# Autodesk Inventor assembly: robot
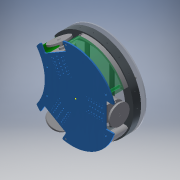
[picture p0: Inventor's stored thumbnail of the model, 180x180]
Saved by Autodesk Inventor 2016 (Build 200138000, 138)
## iProperties
Created: 2015-08-21
Part Number: robot
Document SubType Name: Assembly
Designer: TFHulbert
Author: TFHulbert
## Documents named in this file (11)
- C:\Users\Hulbert Office\Dropbox\SHF Robotics\robot.iam
- C:\Users\Hulbert Office\Dropbox\SHF Robotics\Bottom Plate.ipt
- C:\Users\Hulbert Office\Dropbox\SHF Robotics\Goal.ipt
- C:\Users\Hulbert Office\Dropbox\SHF Robotics\TSOP Plate.ipt
- C:\Users\Hulbert Office\Dropbox\SHF Robotics\motor mount.ipt
- C:\Users\Hulbert Office\Dropbox\SHF Robotics\motor.ipt
- C:\Users\Hulbert Office\Dropbox\SHF Robotics\wheel.ipt
- C:\Users\Hulbert Office\Dropbox\SHF Robotics\small spacer.ipt
- C:\Users\Hulbert Office\Dropbox\SHF Robotics\Middle plate.ipt
- C:\Users\Hulbert Office\Dropbox\SHF Robotics\battery gate.iam
- C:\Users\Hulbert Office\Dropbox\SHF Robotics\battery gate mirrored.iam
## Components (19 placed, 10 different names)
1. Bottom Plate:1 — Mate:1, Mate:4, Mate:5, Mate:6, Mate:7, Mate:8, Mate:9, Mate:24, Mate:25, Mate:26, Mate:27
2. Goal:1 — Mate:1, Mate:2, Mate:3
3. TSOP Plate:1 — Mate:2, Mate:3, Mate:18, Mate:19, Mate:20, Mate:21
4. motor mount:1 — Mate:4, Mate:5, Mate:12
5. motor mount:2 — Mate:6, Mate:8, Mate:10
6. motor mount:3 — Mate:7, Mate:9, Mate:11
7. motor:1 — Mate:11, Mate:14, Insert:2
8. motor:2 — Mate:12, Mate:15, Insert:3
9. motor:3 — Mate:10, Mate:13, Insert:1
10. wheel:1 — Mate:13, Insert:1
11. wheel:2 — Mate:14, Insert:2
12. wheel:3 — Mate:15, Insert:3
13. small spacer:1 — Mate:18
14. small spacer:2 — Mate:19
15. small spacer:3 — Mate:20, Mate:22
16. small spacer:4 — Mate:21, Mate:23
17. Middle plate:1 — Mate:22, Mate:23
18. battery gate:1 [sub-assembly] — Mate:24, Mate:25
19. battery gate mirrored:1 [sub-assembly] — Mate:26, Mate:27
## Relationships (28: Mate 25, Insert 3)
- Mate:1: Bottom Plate:1 ↔ Goal:1
- Mate:2: Goal:1 ↔ TSOP Plate:1
- Mate:3: Goal:1 ↔ TSOP Plate:1
- Mate:4: Bottom Plate:1 ↔ motor mount:1
- Mate:5: Bottom Plate:1 ↔ motor mount:1
- Mate:6: Bottom Plate:1 ↔ motor mount:2
- Mate:7: Bottom Plate:1 ↔ motor mount:3
- Mate:8: Bottom Plate:1 ↔ motor mount:2
- Mate:9: Bottom Plate:1 ↔ motor mount:3
- Mate:10: motor mount:2 ↔ motor:3
- Mate:11: motor mount:3 ↔ motor:1
- Mate:12: motor mount:1 ↔ motor:2
- Mate:13: motor:3 ↔ wheel:1
- Insert:1: motor:3 ↔ wheel:1
- Mate:14: motor:1 ↔ wheel:2
- Insert:2: motor:1 ↔ wheel:2
- Mate:15: motor:2 ↔ wheel:3
- Insert:3: motor:2 ↔ wheel:3
- Mate:18: TSOP Plate:1 ↔ small spacer:1
- Mate:19: TSOP Plate:1 ↔ small spacer:2
- Mate:20: TSOP Plate:1 ↔ small spacer:3
- Mate:21: TSOP Plate:1 ↔ small spacer:4
- Mate:22: small spacer:3 ↔ Middle plate:1
- Mate:23: small spacer:4 ↔ Middle plate:1
- Mate:24: Bottom Plate:1 ↔ battery gate:1
- Mate:25: Bottom Plate:1 ↔ battery gate:1
- Mate:26: Bottom Plate:1 ↔ battery gate mirrored:1
- Mate:27: Bottom Plate:1 ↔ battery gate mirrored:1
